# Autodesk Inventor assembly: BG103_trajan20_21
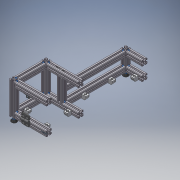
[picture p0: Inventor's stored thumbnail of the model, 180x180]
Saved by Autodesk Inventor 2022.2 (Build 262287000, 287)
## iProperties
Company: HTBLA Kaindorf
RuleStatus: InUse
Created: 2022-08-20
Part Number: BG103_trajan20_21
Project: Zeichenmaschine_v2
Material: Generisch
Description: Gerüst_Step->Bauteil
Document SubType Name: Assembly
Designer: trajan20
AfterDocNew0: iProperties-Editor_aufrufen
Author: jan
Keywords: 2021
## Documents named in this file (7)
- C:\Users\jan\Documents\DrawMachine\DrawMachineConstruction\Projekt\Zeichenmaschine_v2\BG103_trajan20_21_Zeichenmaschine_v2_Gerüst_Step_zu_Bauteil.iam
- C:\Users\jan\Documents\DrawMachine\DrawMachineConstruction\Projekt\Zeichenmaschine_v2\step dateien\gerüst_item_2022-07-24_alu_construct_Projekt_ID-a403a0fdf3734c62922616c2a250de6220_1.ipt
- C:\Users\jan\Documents\DrawMachine\DrawMachineConstruction\Projekt\Zeichenmaschine_v2\step dateien\Magnetschnäpper _093094.ipt
- C:\Users\jan\Documents\DrawMachine\DrawMachineConstruction\Projekt\Zeichenmaschine_v2\step dateien\uniblock_094411m4.ipt
- C:\Users\jan\Documents\DrawMachine\DrawMachineConstruction\Projekt\Zeichenmaschine_v2\step dateien\scharnier_095K2020L00.ipt
- C:\Users\jan\Documents\DrawMachine\DrawMachineConstruction\Projekt\Zeichenmaschine_v2\step dateien\M4_Nutenstein_096214.ipt
- C:\Users\jan\Documents\DrawMachine\DrawMachineConstruction\Projekt\Zeichenmaschine_v2\step dateien\M5_Nutenstein_096215.ipt
## Components (26 placed, 6 different names)
1. gerüst_item_2022-07-24_alu_construct_Projekt_ID-a403a0fdf3734c62922616c2a250de6220_1:1 — Passend:1, Passend:2, Fluchtend:1, Passend:3, Fluchtend:2, Passend:4, Passend:5, Passend:6, Passend:7, Passend:8, Passend:9, Passend:10, Passend:11, Passend:12, Passend:13, Passend:14, Passend:15, Passend:16, Passend:17, Passend:18, Passend:19, Passend:20, Passend:21, Passend:22, Passend:23, Passend:24, Passend:25, Passend:26, Passend:27, Passend:28, Passend:29, Passend:30, Passend:31, Passend:32, Passend:33, Passend:34, Passend:35, Passend:36, Passend:39, Passend:40, Passend:41, Passend:42, Passend:43, Passend:44, Passend:45, Passend:47, Passend:48, Passend:49, Passend:50, Passend:51, Passend:52, Passend:53, Passend:54, Passend:55, Winkel:1, Winkel:2, Passend:57, Winkel:3, Winkel:4
2. Magnetschnäpper _093094:1 — Passend:1, Passend:2, Fluchtend:1, Passend:56, Passend:58
3. Magnetschnäpper _093094:2 — Passend:3, Fluchtend:2, Passend:4
4. uniblock_094411m4:1 — Passend:5, Passend:6
5. uniblock_094411m4:2 — Passend:7, Passend:10, Passend:32
6. uniblock_094411m4:3 — Passend:8, Passend:9, Passend:33
7. uniblock_094411m4:4 — Passend:11, Passend:12, Passend:31
8. uniblock_094411m4:5 — Passend:13, Passend:14
9. uniblock_094411m4:6 — Passend:15, Passend:16
10. uniblock_094411m4:7 — Passend:17, Passend:20
11. uniblock_094411m4:8 — Passend:19, Passend:22
12. uniblock_094411m4:9 — Passend:18, Passend:21
13. uniblock_094411m4:10 — Passend:23, Passend:24, Passend:34
14. uniblock_094411m4:11 — Passend:25, Passend:26, Passend:30
15. uniblock_094411m4:12 — Passend:27, Passend:28, Passend:29
16. scharnier_095K2020L00:1 — Passend:35, Passend:41, Passend:42, Passend:43, Passend:59, Passend:60
17. scharnier_095K2020L00:2 — Passend:36, Passend:39, Passend:40, Passend:44
18. M4_Nutenstein_096214:1 — Passend:45, Winkel:1, Passend:56
19. M4_Nutenstein_096214:3 — Passend:47, Winkel:3, Passend:59
20. M4_Nutenstein_096214:4 — Passend:48, Winkel:4, Passend:60
21. M4_Nutenstein_096214:5 — Passend:49
22. M4_Nutenstein_096214:6 — Passend:50
23. M5_Nutenstein_096215:1 — Passend:51, Passend:54
24. M5_Nutenstein_096215:2 — Passend:52, Passend:53
25. M5_Nutenstein_096215:3 — Passend:55
26. M4_Nutenstein_096214:7 — Winkel:2, Passend:57, Passend:58
## Relationships (63: Mate 57, Angle 4, Flush 2)
- Passend:1 [Mate]: gerüst_item_2022-07-24_alu_construct_Projekt_ID-a403a0fdf3734c62922616c2a250de6220_1:1 ↔ Magnetschnäpper _093094:1
- Passend:2 [Mate] (30 mm): gerüst_item_2022-07-24_alu_construct_Projekt_ID-a403a0fdf3734c62922616c2a250de6220_1:1 ↔ Magnetschnäpper _093094:1
- Fluchtend:1 [Flush] (-1 mm): gerüst_item_2022-07-24_alu_construct_Projekt_ID-a403a0fdf3734c62922616c2a250de6220_1:1 ↔ Magnetschnäpper _093094:1
- Passend:3 [Mate]: gerüst_item_2022-07-24_alu_construct_Projekt_ID-a403a0fdf3734c62922616c2a250de6220_1:1 ↔ Magnetschnäpper _093094:2
- Fluchtend:2 [Flush] (-1 mm): gerüst_item_2022-07-24_alu_construct_Projekt_ID-a403a0fdf3734c62922616c2a250de6220_1:1 ↔ Magnetschnäpper _093094:2
- Passend:4 [Mate] (30 mm): gerüst_item_2022-07-24_alu_construct_Projekt_ID-a403a0fdf3734c62922616c2a250de6220_1:1 ↔ Magnetschnäpper _093094:2
- Passend:5 [Mate]: gerüst_item_2022-07-24_alu_construct_Projekt_ID-a403a0fdf3734c62922616c2a250de6220_1:1 ↔ uniblock_094411m4:1
- Passend:6 [Mate]: gerüst_item_2022-07-24_alu_construct_Projekt_ID-a403a0fdf3734c62922616c2a250de6220_1:1 ↔ uniblock_094411m4:1
- Passend:7 [Mate]: gerüst_item_2022-07-24_alu_construct_Projekt_ID-a403a0fdf3734c62922616c2a250de6220_1:1 ↔ uniblock_094411m4:2
- Passend:8 [Mate]: gerüst_item_2022-07-24_alu_construct_Projekt_ID-a403a0fdf3734c62922616c2a250de6220_1:1 ↔ uniblock_094411m4:3
- Passend:9 [Mate]: gerüst_item_2022-07-24_alu_construct_Projekt_ID-a403a0fdf3734c62922616c2a250de6220_1:1 ↔ uniblock_094411m4:3
- Passend:10 [Mate]: gerüst_item_2022-07-24_alu_construct_Projekt_ID-a403a0fdf3734c62922616c2a250de6220_1:1 ↔ uniblock_094411m4:2
- Passend:11 [Mate]: gerüst_item_2022-07-24_alu_construct_Projekt_ID-a403a0fdf3734c62922616c2a250de6220_1:1 ↔ uniblock_094411m4:4
- Passend:12 [Mate]: gerüst_item_2022-07-24_alu_construct_Projekt_ID-a403a0fdf3734c62922616c2a250de6220_1:1 ↔ uniblock_094411m4:4
- Passend:13 [Mate]: gerüst_item_2022-07-24_alu_construct_Projekt_ID-a403a0fdf3734c62922616c2a250de6220_1:1 ↔ uniblock_094411m4:5
- Passend:14 [Mate]: gerüst_item_2022-07-24_alu_construct_Projekt_ID-a403a0fdf3734c62922616c2a250de6220_1:1 ↔ uniblock_094411m4:5
- Passend:15 [Mate]: gerüst_item_2022-07-24_alu_construct_Projekt_ID-a403a0fdf3734c62922616c2a250de6220_1:1 ↔ uniblock_094411m4:6
- Passend:16 [Mate]: gerüst_item_2022-07-24_alu_construct_Projekt_ID-a403a0fdf3734c62922616c2a250de6220_1:1 ↔ uniblock_094411m4:6
- Passend:17 [Mate]: gerüst_item_2022-07-24_alu_construct_Projekt_ID-a403a0fdf3734c62922616c2a250de6220_1:1 ↔ uniblock_094411m4:7
- Passend:18 [Mate]: gerüst_item_2022-07-24_alu_construct_Projekt_ID-a403a0fdf3734c62922616c2a250de6220_1:1 ↔ uniblock_094411m4:9
- Passend:19 [Mate]: gerüst_item_2022-07-24_alu_construct_Projekt_ID-a403a0fdf3734c62922616c2a250de6220_1:1 ↔ uniblock_094411m4:8
- Passend:20 [Mate]: gerüst_item_2022-07-24_alu_construct_Projekt_ID-a403a0fdf3734c62922616c2a250de6220_1:1 ↔ uniblock_094411m4:7
- Passend:21 [Mate]: gerüst_item_2022-07-24_alu_construct_Projekt_ID-a403a0fdf3734c62922616c2a250de6220_1:1 ↔ uniblock_094411m4:9
- Passend:22 [Mate]: gerüst_item_2022-07-24_alu_construct_Projekt_ID-a403a0fdf3734c62922616c2a250de6220_1:1 ↔ uniblock_094411m4:8
- Passend:23 [Mate]: gerüst_item_2022-07-24_alu_construct_Projekt_ID-a403a0fdf3734c62922616c2a250de6220_1:1 ↔ uniblock_094411m4:10
- Passend:24 [Mate]: gerüst_item_2022-07-24_alu_construct_Projekt_ID-a403a0fdf3734c62922616c2a250de6220_1:1 ↔ uniblock_094411m4:10
- Passend:25 [Mate]: gerüst_item_2022-07-24_alu_construct_Projekt_ID-a403a0fdf3734c62922616c2a250de6220_1:1 ↔ uniblock_094411m4:11
- Passend:26 [Mate]: gerüst_item_2022-07-24_alu_construct_Projekt_ID-a403a0fdf3734c62922616c2a250de6220_1:1 ↔ uniblock_094411m4:11
- Passend:27 [Mate]: gerüst_item_2022-07-24_alu_construct_Projekt_ID-a403a0fdf3734c62922616c2a250de6220_1:1 ↔ uniblock_094411m4:12
- Passend:28 [Mate]: gerüst_item_2022-07-24_alu_construct_Projekt_ID-a403a0fdf3734c62922616c2a250de6220_1:1 ↔ uniblock_094411m4:12
- Passend:29 [Mate] (60 mm): gerüst_item_2022-07-24_alu_construct_Projekt_ID-a403a0fdf3734c62922616c2a250de6220_1:1 ↔ uniblock_094411m4:12
- Passend:30 [Mate] (60 mm): gerüst_item_2022-07-24_alu_construct_Projekt_ID-a403a0fdf3734c62922616c2a250de6220_1:1 ↔ uniblock_094411m4:11
- Passend:31 [Mate] (40 mm): gerüst_item_2022-07-24_alu_construct_Projekt_ID-a403a0fdf3734c62922616c2a250de6220_1:1 ↔ uniblock_094411m4:4
- Passend:32 [Mate] (60 mm): gerüst_item_2022-07-24_alu_construct_Projekt_ID-a403a0fdf3734c62922616c2a250de6220_1:1 ↔ uniblock_094411m4:2
- Passend:33 [Mate] (60 mm): gerüst_item_2022-07-24_alu_construct_Projekt_ID-a403a0fdf3734c62922616c2a250de6220_1:1 ↔ uniblock_094411m4:3
- Passend:34 [Mate] (50 mm): gerüst_item_2022-07-24_alu_construct_Projekt_ID-a403a0fdf3734c62922616c2a250de6220_1:1 ↔ uniblock_094411m4:10
- Passend:35 [Mate]: gerüst_item_2022-07-24_alu_construct_Projekt_ID-a403a0fdf3734c62922616c2a250de6220_1:1 ↔ scharnier_095K2020L00:1
- Passend:36 [Mate] (2.5 mm): gerüst_item_2022-07-24_alu_construct_Projekt_ID-a403a0fdf3734c62922616c2a250de6220_1:1 ↔ scharnier_095K2020L00:2
- Passend:39 [Mate]: gerüst_item_2022-07-24_alu_construct_Projekt_ID-a403a0fdf3734c62922616c2a250de6220_1:1 ↔ scharnier_095K2020L00:2
- Passend:40 [Mate] (2.5 mm): gerüst_item_2022-07-24_alu_construct_Projekt_ID-a403a0fdf3734c62922616c2a250de6220_1:1 ↔ scharnier_095K2020L00:2
- Passend:41 [Mate] (2.5 mm): gerüst_item_2022-07-24_alu_construct_Projekt_ID-a403a0fdf3734c62922616c2a250de6220_1:1 ↔ scharnier_095K2020L00:1
- Passend:42 [Mate] (2.5 mm): gerüst_item_2022-07-24_alu_construct_Projekt_ID-a403a0fdf3734c62922616c2a250de6220_1:1 ↔ scharnier_095K2020L00:1
- Passend:43 [Mate] (30 mm): gerüst_item_2022-07-24_alu_construct_Projekt_ID-a403a0fdf3734c62922616c2a250de6220_1:1 ↔ scharnier_095K2020L00:1
- Passend:44 [Mate] (30 mm): gerüst_item_2022-07-24_alu_construct_Projekt_ID-a403a0fdf3734c62922616c2a250de6220_1:1 ↔ scharnier_095K2020L00:2
- Passend:45 [Mate]: gerüst_item_2022-07-24_alu_construct_Projekt_ID-a403a0fdf3734c62922616c2a250de6220_1:1 ↔ M4_Nutenstein_096214:1
- Passend:47 [Mate]: gerüst_item_2022-07-24_alu_construct_Projekt_ID-a403a0fdf3734c62922616c2a250de6220_1:1 ↔ M4_Nutenstein_096214:3
- Passend:48 [Mate]: gerüst_item_2022-07-24_alu_construct_Projekt_ID-a403a0fdf3734c62922616c2a250de6220_1:1 ↔ M4_Nutenstein_096214:4
- Passend:49 [Mate]: gerüst_item_2022-07-24_alu_construct_Projekt_ID-a403a0fdf3734c62922616c2a250de6220_1:1 ↔ M4_Nutenstein_096214:5
- Passend:50 [Mate]: gerüst_item_2022-07-24_alu_construct_Projekt_ID-a403a0fdf3734c62922616c2a250de6220_1:1 ↔ M4_Nutenstein_096214:6
- Passend:51 [Mate]: gerüst_item_2022-07-24_alu_construct_Projekt_ID-a403a0fdf3734c62922616c2a250de6220_1:1 ↔ M5_Nutenstein_096215:1
- Passend:52 [Mate]: gerüst_item_2022-07-24_alu_construct_Projekt_ID-a403a0fdf3734c62922616c2a250de6220_1:1 ↔ M5_Nutenstein_096215:2
- Passend:53 [Mate] (2.5 mm): gerüst_item_2022-07-24_alu_construct_Projekt_ID-a403a0fdf3734c62922616c2a250de6220_1:1 ↔ M5_Nutenstein_096215:2
- Passend:54 [Mate] (2.5 mm): gerüst_item_2022-07-24_alu_construct_Projekt_ID-a403a0fdf3734c62922616c2a250de6220_1:1 ↔ M5_Nutenstein_096215:1
- Passend:55 [Mate]: gerüst_item_2022-07-24_alu_construct_Projekt_ID-a403a0fdf3734c62922616c2a250de6220_1:1 ↔ M5_Nutenstein_096215:3
- Winkel:1 [Angle] (180 deg): gerüst_item_2022-07-24_alu_construct_Projekt_ID-a403a0fdf3734c62922616c2a250de6220_1:1 ↔ M4_Nutenstein_096214:1
- Passend:56 [Mate]: Magnetschnäpper _093094:1 ↔ M4_Nutenstein_096214:1
- Winkel:2 [Angle] (0 deg): gerüst_item_2022-07-24_alu_construct_Projekt_ID-a403a0fdf3734c62922616c2a250de6220_1:1 ↔ M4_Nutenstein_096214:7
- Passend:57 [Mate]: gerüst_item_2022-07-24_alu_construct_Projekt_ID-a403a0fdf3734c62922616c2a250de6220_1:1 ↔ M4_Nutenstein_096214:7
- Passend:58 [Mate]: Magnetschnäpper _093094:1 ↔ M4_Nutenstein_096214:7
- Winkel:3 [Angle] (0 deg): gerüst_item_2022-07-24_alu_construct_Projekt_ID-a403a0fdf3734c62922616c2a250de6220_1:1 ↔ M4_Nutenstein_096214:3
- Passend:59 [Mate]: scharnier_095K2020L00:1 ↔ M4_Nutenstein_096214:3
- Winkel:4 [Angle] (0 deg): gerüst_item_2022-07-24_alu_construct_Projekt_ID-a403a0fdf3734c62922616c2a250de6220_1:1 ↔ M4_Nutenstein_096214:4
- Passend:60 [Mate]: scharnier_095K2020L00:1 ↔ M4_Nutenstein_096214:4
